# Autodesk Inventor assembly: Assembly_newholders
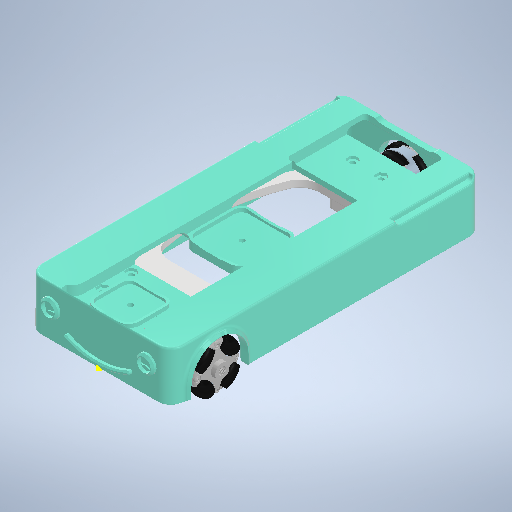
[picture p0: Inventor's stored thumbnail of the model, 512x512]
Saved by Autodesk Inventor 2025 (Build 290162000, 162)
## iProperties
Created: 2024-07-05
Part Number: Assembly_newholders
Document SubType Name: Assembly
Designer: Pintu
Author: Pintu
## Documents named in this file (5)
- D:\CMC\my_inventor\ArmBo_v2\wearable\Assembly_newholders.iam
- D:\CMC\my_inventor\ArmBo_v2\wearable\chasis.ipt
- D:\CMC\my_inventor\ArmBo_v2\wearable\wearable.ipt
- D:\CMC\my_inventor\ArmBo_v2\wearable\wheel_holder_strong.ipt
- D:\CMC\my_inventor\ArmBo_v2\wheels\omniwheel_38mm\omniwheel_38mm\wheel_38mm_assembly.iam
## Components (6 placed, 4 different names)
1. chasis:1 — Mate:1, Flush:1, Mate:2, Mate:3, Flush:2, Mate:10
2. wearable:1 — Mate:1, Flush:1, Mate:2
3. wheel_holder_strong:1 — Mate:3, Flush:2, Mate:4, Mate:5, Mate:6, Mate:7, Mate:8, Mate:9, Mate:10
4. wheel_38mm_assembly:1 [sub-assembly] — Mate:6, Mate:7
5. wheel_38mm_assembly:2 [sub-assembly] — Mate:4, Mate:5
6. wheel_38mm_assembly:3 [sub-assembly] — Mate:8, Mate:9
## Relationships (12: Mate 10, Flush 2)
- Mate:1: chasis:1 ↔ wearable:1
- Flush:1: chasis:1 ↔ wearable:1
- Mate:2 (0.4 mm): chasis:1 ↔ wearable:1
- Mate:3: chasis:1 ↔ wheel_holder_strong:1
- Flush:2 (2 mm): chasis:1 ↔ wheel_holder_strong:1
- Mate:4: wheel_holder_strong:1 ↔ wheel_38mm_assembly:2
- Mate:5: wheel_holder_strong:1 ↔ wheel_38mm_assembly:2
- Mate:6: wheel_holder_strong:1 ↔ wheel_38mm_assembly:1
- Mate:7: wheel_holder_strong:1 ↔ wheel_38mm_assembly:1
- Mate:8: wheel_holder_strong:1 ↔ wheel_38mm_assembly:3
- Mate:9: wheel_holder_strong:1 ↔ wheel_38mm_assembly:3
- Mate:10: chasis:1 ↔ wheel_holder_strong:1
